# Autodesk Inventor assembly: estop v2
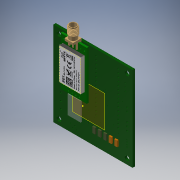
[picture p0: Inventor's stored thumbnail of the model, 180x180]
Saved by Autodesk Inventor 2019 (Build 230136000, 136)
## iProperties
Created: 2019-10-02
Part Number: estop v2
Document SubType Name: Assembly
Designer: rybit
Author: rybit
## Documents named in this file (5)
- I:\CMR4GR\Documents\Inventor\ESTOP V2\estop v2.iam
- I:\CMR4GR\Documents\Inventor\ESTOP V2\estop v2.brd_Outline.ipt
- I:\CMR4GR\Documents\Inventor\ESTOP V2\E01-ML01DP5, E01-ML01DP5_23.ipt
- I:\CMR4GR\Documents\Inventor\ESTOP V2\sma.ipt
- I:\CMR4GR\Documents\Inventor\ESTOP V2\pin header.iam
## Components (15 placed, 4 different names)
1. estop v2.brd_Outline:1 — Mate:15, Mate:16, Angle:1
2. U_1_24 — Mate:1, Mate:2, Flush:1, Mate:12, Mate:13, Mate:14, Flush:20, Flush:21, Flush:22, Flush:23, Flush:24, Flush:25, Mate:16, Angle:1
3. sma:1 — Mate:1, Mate:2, Flush:1
4. pin header:5 [sub-assembly] — Mate:5, Flush:6, Flush:7
5. pin header:6 [sub-assembly] — Mate:5, Flush:6, Flush:7, Mate:6, Flush:8, Flush:9
6. pin header:7 [sub-assembly] — Mate:6, Flush:8, Flush:9, Mate:7, Flush:10, Flush:11
7. pin header:8 [sub-assembly] — Mate:7, Flush:10, Flush:11, Mate:11, Flush:18, Flush:19
8. pin header:11 [sub-assembly] — Mate:3, Flush:2, Flush:3, Mate:13, Flush:22, Mate:15
9. pin header:12 [sub-assembly] — Mate:3, Flush:2, Flush:3, Flush:21
10. pin header:13 [sub-assembly]
11. pin header:14 [sub-assembly] — Mate:14, Flush:20, Flush:23
12. pin header:15 [sub-assembly] — Flush:24
13. pin header:16 [sub-assembly] — Flush:25
14. pin header:17 [sub-assembly]
15. pin header:18 [sub-assembly] — Mate:11, Flush:18, Flush:19, Mate:12
## Relationships (42: Flush 25, Mate 16, Angle 1)
- Mate:1: U_1_24 ↔ sma:1
- Mate:2: U_1_24 ↔ sma:1
- Flush:1 (6.0579 mm): U_1_24 ↔ sma:1
- Mate:3: pin header:11 ↔ pin header:12
- Flush:2: pin header:11 ↔ pin header:12
- Flush:3: pin header:11 ↔ pin header:12
- [Mate]: pin header:13 ↔ pin header:14
- [Flush]: pin header:13 ↔ pin header:14
- [Flush]: pin header:13 ↔ pin header:14
- Mate:5: pin header:5 ↔ pin header:6
- Flush:6: pin header:5 ↔ pin header:6
- Flush:7: pin header:5 ↔ pin header:6
- Mate:6: pin header:6 ↔ pin header:7
- Flush:8: pin header:6 ↔ pin header:7
- Flush:9: pin header:6 ↔ pin header:7
- Mate:7: pin header:7 ↔ pin header:8
- Flush:10: pin header:7 ↔ pin header:8
- Flush:11: pin header:7 ↔ pin header:8
- [Mate]: pin header:15 ↔ pin header:16
- [Flush]: pin header:15 ↔ pin header:16
- [Flush]: pin header:15 ↔ pin header:16
- [Mate]: pin header:16 ↔ pin header:17
- [Flush]: pin header:16 ↔ pin header:17
- [Flush]: pin header:16 ↔ pin header:17
- [Mate]: pin header:17 ↔ pin header:18
- [Flush]: pin header:17 ↔ pin header:18
- [Flush]: pin header:17 ↔ pin header:18
- Mate:11: pin header:8 ↔ pin header:18
- Flush:18: pin header:8 ↔ pin header:18
- Flush:19: pin header:8 ↔ pin header:18
- Mate:12: U_1_24 ↔ pin header:18
- Mate:13: U_1_24 ↔ pin header:11
- Mate:14: U_1_24 ↔ pin header:14
- Flush:20 (1.27 mm): U_1_24 ↔ pin header:14
- Flush:21 (1.27 mm): U_1_24 ↔ pin header:12
- Flush:22 (0.508 mm): U_1_24 ↔ pin header:11
- Flush:23 (0.508 mm): U_1_24 ↔ pin header:14
- Flush:24 (3.9878 mm): U_1_24 ↔ pin header:15
- Flush:25 (0.2794 mm): U_1_24 ↔ pin header:16
- Mate:15: estop v2.brd_Outline:1 ↔ pin header:11
- Mate:16: estop v2.brd_Outline:1 ↔ U_1_24
- Angle:1 (0 deg): estop v2.brd_Outline:1 ↔ U_1_24
## Named parameters: d8_d5 = 0 mm, d9_d6 = 0 mm, d10_d7 = 0 mm, d20_d13 = 0 mm, d21_d14 = 0 mm, d22_d15 = 0 mm, d23_d16 = 0 mm, d24_d17 = 0 mm, d25_d18 = 0 mm, d26_d19 = 0 mm, d27_d11 = 0 mm, d28_d12 = 0 mm
